# Autodesk Inventor assembly: 536236 ADN-20-15-A-P-A---(asm_0)
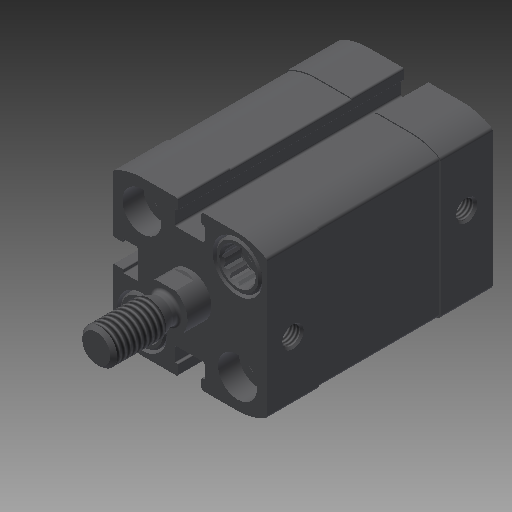
[picture p0: Inventor's stored thumbnail of the model, 512x512]
Saved by Autodesk Inventor 2017 (Build 210142000, 142)
## iProperties
Category: PARTsolutions
Company: FESTO
Created: 2018-05-29
Part Number: 536236 ADN-20-15-A-P-A---(asm_0)
Catalog Web Link: www.cadenas.de
Description: ADN-Compact cylinder
Vendor: FESTO
Document SubType Name: Assembly
Designer: psAdmin
Manufacturer: FESTO
Mass: 163 g
PSOL_IDENT_0: {$CADENAS_DATA\23d-libs\festo\parts\a\adn\adn_std_tab.prj},213 {VTYP=3D},{STYP=ASSTAB},{NB=536236 AD
PSOL_IDENT_1: N-20-15-A-P-A---(asm_0)},{LINA=536236 ADN-20-15-A-P-A},{NN=ADN},{DATE=17.05.2018 10:40:18},{GEOMDATE=
PSOL_IDENT_2: 24.04.2017 11:47:47},{VERSION=},{LINEID=280},{LINESUBID=-1},{WBVAR=HUBST}  {NB=536236 ADN-20-15-A-P-
PSOL_IDENT_3: A---(asm_0)},{LINA=536236 ADN-20-15-A-P-A},{KT=DUMMY},{TNR=536236},{TYP=ADN-20-15-A-P-A},{KDM=20},{H
PSOL_IDENT_4: UB=15},{HUBST=0},{DF=P},{TH=A},{Q=0},{S2=0},{K2=0},{K5=0},{K8=0},{ZZ=0},{A=16.000},{AF=14.000},{BG=1
PSOL_IDENT_5: 9.500},{D1=9.000},{D5=9.000},{E=35.500},{EE=M5},{EEN=5.000},{EEK=4.019},{G=12.000},{KF=M6},{KFN=6.00
PSOL_IDENT_6: 0},{KFK=4.917},{KFNW=6},{KFKW=4.917},{KK=M8},{KKN=8.000},{KKK=6.466},{KKNW=8},{KKKW=6.466},{L3=5.000
PSOL_IDENT_7: },{L12=4.200},{MM=10.000},{PL=6.000},{RR=4.100},{RT=M5},{RTN=5.000},{RTK=4.134},{SW=9.000},{T1=2.100
PSOL_IDENT_8: },{T4=2.600},{TG=22.000},{WH=5.500},{ZA=37.000},{ZB=42.500},{J3=2.600},{SWQ=9.000},{RA=0.000},{RU=23
PSOL_IDENT_9: .800},{RT1=3.400},{RB1=5.400},{RB2=6.800},{R1=12.750},{R2=0.800},{FORM=1},{MASSBKS=0.030},{MASSHKS=0
PSOL_IDENT_10: .006},{MASSBZR=0.131},{MASSHZR=0.021},{CNSMASSEXACT=0.1625},{PPATH=assemblies/adn_asmtpl.prj}
NN: ADN
NT: Compact cylinder
NB: 536236 ADN-20-15-A-P-A---(asm_0)
NBSYN: $TNR. $TYP.---(asm_$HUBST.)
LINA: 536236 ADN-20-15-A-P-A
OFFICIAL_STANDARD_NUMBERS: ISO 21287
TNR: 536236
TYP: ADN-20-15-A-P-A
KDM: 20
HUB: 15
HUBST: 0
DF: P
TH: A
A: 16.000
AF: 14.000
BG: 19.500
D1: 9.000
D5: 9.000
E: 35.500
EE: M5
G: 12.000
KF: M6
KK: M8
L3: 5.000
L12: 4.200
MM: 10.000
PL: 6.000
RR: 4.100
RT: M5
SW: 9.000
T1: 2.100
T4: 2.600
TG: 22.000
WH: 5.500
ZA: 37.000
ZB: 42.500
J3: 2.600
RA: 0.000
RU: 23.800
R1: 12.750
R2: 0.800
CNSMASSEXACT: 0.163
SUPPLIER: FESTO
ARTICLENO: 536236 ADN-20-15-A-P-A---(asm_0)
BOMINFO: 536236 ADN-20-15-A-P-A
CREATOR: CADENAS GmbH
Title: 536236 ADN-20-15-A-P-A
Author: Cadenas PARTsolutions
Comments: Compact cylinder
## Documents named in this file (3)
- C:\Users\Pies\Desktop\Rzeczy\AGH\Semestr 2\ZIPK\Chwytak\Moj_Chwd_Pytak\Inventorowe chwytaki\Silownik\536236 ADN-20-15-A-P-A---(asm_0).iam
- C:\Users\Pies\Desktop\Rzeczy\AGH\Semestr 2\ZIPK\Chwytak\Moj_Chwd_Pytak\Inventorowe chwytaki\Silownik\536233 ADN-15-P---(Z).ipt
- C:\Users\Pies\Desktop\Rzeczy\AGH\Semestr 2\ZIPK\Chwytak\Moj_Chwd_Pytak\Inventorowe chwytaki\Silownik\536233 ADN-15-P-A_(KS).ipt
## Components (2 placed, 2 different names)
1. 536233 ADN-15-P---(Z):1 — CYLINDER_Z@1 <-> PISTON_Z@2, CYLINDER_YZ@1 <-> PISTON_YZ@2
2. 536233 ADN-15-P-A_(KS):1 — CYLINDER_Z@1 <-> PISTON_Z@2, CYLINDER_YZ@1 <-> PISTON_YZ@2
## Relationships (2: Mate 1, Angle 1)
- CYLINDER_Z@1 <-> PISTON_Z@2 [Mate]: 536233 ADN-15-P---(Z):1 ↔ 536233 ADN-15-P-A_(KS):1
- CYLINDER_YZ@1 <-> PISTON_YZ@2 [Angle] (0 deg): 536233 ADN-15-P---(Z):1 ↔ 536233 ADN-15-P-A_(KS):1
